# Autodesk Inventor assembly: MaskAss
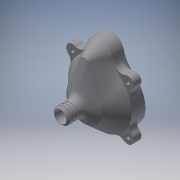
[picture p0: Inventor's stored thumbnail of the model, 180x180]
Saved by Autodesk Inventor 2018 (Build 220112000, 112)
## iProperties
Created: 2020-03-23
Part Number: MaskAss
Document SubType Name: Assembly
Designer: emile
Author: emile
## Documents named in this file (3)
- C:\Users\emile\OneDrive\Documents\Inventor\Respirator\MaskAss.iam
- C:\Users\emile\OneDrive\Documents\Inventor\Respirator\Mask.ipt
- C:\Users\emile\OneDrive\Documents\Inventor\Respirator\Mask2.ipt
## Components (2 placed, 2 different names)
1. Mask:1 — Mate:1, Mate:2, Mate:3
2. Mask2:1 — Mate:1, Mate:2, Mate:3
## Relationships (3: Mate 3)
- Mate:1: Mask:1 ↔ Mask2:1
- Mate:2: Mask:1 ↔ Mask2:1
- Mate:3: Mask:1 ↔ Mask2:1
